# Autodesk Inventor assembly: Подъёмник
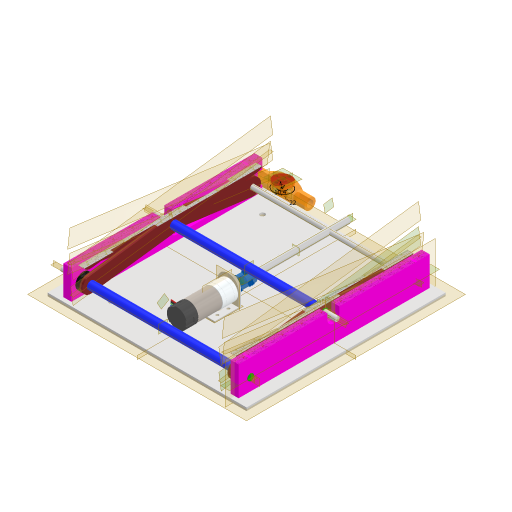
[picture p0: Inventor's stored thumbnail of the model, 512x512]
Saved by Autodesk Inventor 2023.2 (Build 272271030, 271C)
## iProperties
Created: 2025-03-18
Part Number: Подъёмник
Document SubType Name: Assembly
Designer: Коноваленко
Author: Коноваленко
## Documents named in this file (18)
- D:\!Rover\Rover\Rover_construction\Подъёмник.iam
- D:\!Rover\Rover\Rover_construction\Платформа подъёмника.ipt
- D:\!Rover\Rover\Rover_construction\Рельс платформы подъёмника.ipt
- D:\!Rover\Rover\Rover_construction\Рычаг платформы подъёмника.ipt
- D:\!Rover\Rover\Rover_construction\Основание подъёмника.ipt
- D:\!Rover\Rover\Rover_construction\Трубка.ipt
- D:\!Rover\Rover\Rover_construction\Рельс платформы подъёмника_MIR.ipt
- D:\!Rover\Rover\Rover_construction\Бабышка.ipt
- D:\!Rover\Rover\Rover_construction\Рельс платформы подъёмника_MIR1.ipt
- D:\!Rover\Rover\Rover_construction\Трубка основания.ipt
- D:\!Rover\Rover\Rover_construction\Подшипник.ipt
- D:\!Rover\Rover\Rover_construction\шпилька 6мм.ipt
- D:\!Rover\Rover\Rover_construction\Уголок крепления мотора.ipt
- D:\!Rover\Rover\Rover_construction\25d-metal-gearmotor-20.4-encoder.ipt
- D:\!Rover\Rover\Rover_construction\ftulka.ipt
- D:\!Rover\Rover\Rover_construction\Трапециевидный винт.ipt
- D:\!Rover\Rover\Rover_construction\Крепление ходовой гайки.ipt
- D:\!Rover\Rover\Rover_construction\THSL-300-8D õîäîâàÿ ãàéêà.ipt
## Components (53 placed, 17 different names)
1. Платформа подъёмника:1 — Совмещение:4, Заподлицо:4, Заподлицо:5, Заподлицо:10, Заподлицо:11, Совмещение:15
2. Рельс платформы подъёмника:1 — Совмещение:4, Заподлицо:4, Заподлицо:5, С поворотом:48, С поворотом:59
3. Основание подъёмника:1 — Совмещение:9, Заподлицо:8, Заподлицо:9, Заподлицо:12, Заподлицо:13, Совмещение:16, Совмещение:17, Заподлицо:14, Заподлицо:15, Совмещение:44, Заподлицо:21
4. Рельс платформы подъёмника:4 — Совмещение:9, Заподлицо:8, Заподлицо:9, С поворотом:32, Ползун:3, С поворотом:45, Совмещение:53
5. Трубка:1 — Жесткий:1, С поворотом:40, Совмещение:20, Совмещение:36, Заподлицо:16
6. Трубка:2 — С поворотом:38, С поворотом:39, Совмещение:18, Совмещение:39, Заподлицо:19
7. Рельс платформы подъёмника_MIR:1 — Заподлицо:10, Заподлицо:11, Совмещение:15, С поворотом:47, Ползун:5, Совмещение:53
8. Рельс платформы подъёмника_MIR1:1 — Заподлицо:12, Заподлицо:13, Совмещение:16, С поворотом:33, Ползун:4, С поворотом:46
9. Бабышка:9 — С поворотом:33, С поворотом:34
10. Бабышка:10 — С поворотом:32, С поворотом:37
11. Трубка основания:1 — Совмещение:30, Совмещение:31
12. Трубка основания:2 — Совмещение:18, Совмещение:19
13. Подшипник:1 — Ползун:5, С поворотом:55
14. Подшипник:2 — С поворотом:57
15. Подшипник:3 — Ползун:3, С поворотом:50
16. Подшипник:4 — Ползун:4, С поворотом:51
17. Трубка основания:3 — Совмещение:20, Совмещение:21
18. Трубка:3 — С поворотом:41, С поворотом:42, Совмещение:22, Совмещение:37, Заподлицо:17
19. Трубка:5 — С поворотом:43, С поворотом:44, Совмещение:24, Совмещение:38, Заподлицо:18
20. Трубка основания:4 — Совмещение:22, Совмещение:23
21. Трубка основания:5 — Совмещение:24, Совмещение:25
22. Трубка:6 — С поворотом:47, С поворотом:48, С поворотом:54
23. Трубка:7 — С поворотом:45, С поворотом:46, Совмещение:26, Совмещение:40, Заподлицо:20
24. Трубка основания:6 — Совмещение:28, Совмещение:29
25. Трубка основания:7 — Совмещение:26, Совмещение:27
26. шпилька 6мм:1 — С поворотом:50, С поворотом:51, С поворотом:52
27. Трубка:8 — С поворотом:52, С поворотом:53, Совмещение:28
28. Трубка:9 — С поворотом:56, С поворотом:58, Совмещение:30
29. шпилька 6мм:3 — С поворотом:55, С поворотом:56, С поворотом:57
30. Трубка:10 — С поворотом:59, Совмещение:32, Совмещение:35
31. Трубка основания:8 — Совмещение:32, Совмещение:33, Совмещение:34
32. Бабышка:11 — С поворотом:60
33. Бабышка:12 — С поворотом:61
34. шпилька 6мм:4 — Совмещение:37, Заподлицо:17
35. шпилька 6мм:5 — Совмещение:40, Заподлицо:20
36. шпилька 6мм:6 — Совмещение:38, Заподлицо:18
37. шпилька 6мм:7 — Совмещение:36, Заподлицо:16
38. шпилька 6мм:8 — Совмещение:34, Совмещение:35
39. шпилька 6мм:9 — Совмещение:39, Заподлицо:19
40. Уголок крепления мотора:1 — Совмещение:44, Заподлицо:21, Совмещение:45, Совмещение:46, Совмещение:47, Совмещение:52
41. 25d-metal-gearmotor-20.4-encoder:1 — Совмещение:45, Совмещение:46, Совмещение:47, Совмещение:49
42. ftulka:1 — Совмещение:49, Совмещение:50, Совмещение:51, Совмещение:52
43. Трапециевидный винт:6 — Совмещение:50, Совмещение:51
44. Крепление ходовой гайки:1 — Совмещение:54, Совмещение:55
45. THSL-300-8D õîäîâàÿ ãàéêà:1 — Совмещение:54, Совмещение:55
46. Рычаг платформы подъёмника:1 — С поворотом:11, С поворотом:36, С поворотом:37
47. Рычаг платформы подъёмника:2 — С поворотом:11, С поворотом:35, Жесткий:1, С поворотом:42, С поворотом:54
48. Рычаг платформы подъёмника:3 — С поворотом:8, С поворотом:17, Совмещение:21, Совмещение:25, Совмещение:31, С поворотом:61
49. Рычаг платформы подъёмника:4 — С поворотом:8, С поворотом:15, С поворотом:40, С поворотом:41, Совмещение:33
50. Рычаг платформы подъёмника:5 — С поворотом:12, С поворотом:35, С поворотом:58, С поворотом:60
51. Рычаг платформы подъёмника:6 — С поворотом:12, С поворотом:36, С поворотом:39, С поворотом:44, С поворотом:53
52. Рычаг платформы подъёмника:7 — С поворотом:16, С поворотом:17, С поворотом:38, С поворотом:43, Совмещение:29
53. Рычаг платформы подъёмника:8 — С поворотом:15, С поворотом:16, С поворотом:34, Совмещение:19, Совмещение:23, Совмещение:27
## Relationships (94: Mate 39, RevoluteJoint 35, Flush 16, TranslationJoint 3, WeldJoint 1)
- Совмещение:4 [Mate]: Платформа подъёмника:1 ↔ Рельс платформы подъёмника:1
- Совмещение:9 [Mate]: Основание подъёмника:1 ↔ Рельс платформы подъёмника:4
- Заподлицо:4 [Flush] (5 mm): Платформа подъёмника:1 ↔ Рельс платформы подъёмника:1
- Заподлицо:5 [Flush] (15 mm): Платформа подъёмника:1 ↔ Рельс платформы подъёмника:1
- Заподлицо:8 [Flush] (5 mm): Основание подъёмника:1 ↔ Рельс платформы подъёмника:4
- Заподлицо:9 [Flush] (15 mm): Основание подъёмника:1 ↔ Рельс платформы подъёмника:4
- Заподлицо:10 [Flush] (5 mm): Платформа подъёмника:1 ↔ Рельс платформы подъёмника_MIR:1
- Заподлицо:11 [Flush] (15 mm): Платформа подъёмника:1 ↔ Рельс платформы подъёмника_MIR:1
- Совмещение:15 [Mate]: Платформа подъёмника:1 ↔ Рельс платформы подъёмника_MIR:1
- С поворотом:8 [RevoluteJoint]: Рычаг платформы подъёмника:3 ↔ Рычаг платформы подъёмника:4
- С поворотом:11 [RevoluteJoint]: Рычаг платформы подъёмника:1 ↔ Рычаг платформы подъёмника:2
- С поворотом:12 [RevoluteJoint]: Рычаг платформы подъёмника:5 ↔ Рычаг платформы подъёмника:6
- С поворотом:15 [RevoluteJoint]: Рычаг платформы подъёмника:4 ↔ Рычаг платформы подъёмника:8
- С поворотом:16 [RevoluteJoint]: Рычаг платформы подъёмника:7 ↔ Рычаг платформы подъёмника:8
- С поворотом:17 [RevoluteJoint]: Рычаг платформы подъёмника:3 ↔ Рычаг платформы подъёмника:7
- Заподлицо:12 [Flush] (5 mm): Основание подъёмника:1 ↔ Рельс платформы подъёмника_MIR1:1
- Заподлицо:13 [Flush] (15 mm): Основание подъёмника:1 ↔ Рельс платформы подъёмника_MIR1:1
- Совмещение:16 [Mate]: Основание подъёмника:1 ↔ Рельс платформы подъёмника_MIR1:1
- Совмещение:17 [Mate]: Основание подъёмника:1
- Заподлицо:14 [Flush]: Основание подъёмника:1
- Заподлицо:15 [Flush]: Основание подъёмника:1
- С поворотом:32 [RevoluteJoint]: Рельс платформы подъёмника:4 ↔ Бабышка:10
- С поворотом:33 [RevoluteJoint]: Рельс платформы подъёмника_MIR1:1 ↔ Бабышка:9
- С поворотом:34 [RevoluteJoint]: Бабышка:9 ↔ Рычаг платформы подъёмника:8
- С поворотом:35 [RevoluteJoint]: Рычаг платформы подъёмника:2 ↔ Рычаг платформы подъёмника:5
- С поворотом:36 [RevoluteJoint]: Рычаг платформы подъёмника:1 ↔ Рычаг платформы подъёмника:6
- С поворотом:37 [RevoluteJoint]: Бабышка:10 ↔ Рычаг платформы подъёмника:1
- С поворотом:38 [RevoluteJoint] (-0.5 mm): Трубка:2 ↔ Рычаг платформы подъёмника:7
- С поворотом:39 [RevoluteJoint] (0.5 mm): Трубка:2 ↔ Рычаг платформы подъёмника:6
- Жесткий:1 [WeldJoint] (0.5 mm): Трубка:1 ↔ Рычаг платформы подъёмника:2
- С поворотом:40 [RevoluteJoint] (0.5 mm): Трубка:1 ↔ Рычаг платформы подъёмника:4
- Ползун:3 [TranslationJoint]: Рельс платформы подъёмника:4 ↔ Подшипник:3
- Ползун:4 [TranslationJoint]: Рельс платформы подъёмника_MIR1:1 ↔ Подшипник:4
- Совмещение:18 [Mate]: Трубка:2 ↔ Трубка основания:2
- Совмещение:19 [Mate] (0.5 mm): Трубка основания:2 ↔ Рычаг платформы подъёмника:8
- Совмещение:20 [Mate]: Трубка:1 ↔ Трубка основания:3
- Совмещение:21 [Mate] (0.5 mm): Трубка основания:3 ↔ Рычаг платформы подъёмника:3
- С поворотом:41 [RevoluteJoint] (0.5 mm): Трубка:3 ↔ Рычаг платформы подъёмника:4
- С поворотом:42 [RevoluteJoint] (-0.5 mm): Трубка:3 ↔ Рычаг платформы подъёмника:2
- С поворотом:43 [RevoluteJoint] (-0.5 mm): Трубка:5 ↔ Рычаг платформы подъёмника:7
- С поворотом:44 [RevoluteJoint] (-0.5 mm): Трубка:5 ↔ Рычаг платформы подъёмника:6
- Совмещение:22 [Mate]: Трубка:3 ↔ Трубка основания:4
- Совмещение:23 [Mate] (0.5 mm): Трубка основания:4 ↔ Рычаг платформы подъёмника:8
- Совмещение:24 [Mate]: Трубка:5 ↔ Трубка основания:5
- Совмещение:25 [Mate] (0.5 mm): Трубка основания:5 ↔ Рычаг платформы подъёмника:3
- С поворотом:45 [RevoluteJoint] (0.5 mm): Рельс платформы подъёмника:4 ↔ Трубка:7
- С поворотом:46 [RevoluteJoint] (0.5 mm): Рельс платформы подъёмника_MIR1:1 ↔ Трубка:7
- Совмещение:26 [Mate]: Трубка:7 ↔ Трубка основания:7
- Совмещение:27 [Mate] (0.5 mm): Трубка основания:7 ↔ Рычаг платформы подъёмника:8
- С поворотом:47 [RevoluteJoint] (0.5 mm): Рельс платформы подъёмника_MIR:1 ↔ Трубка:6
- С поворотом:48 [RevoluteJoint] (-0.5 mm): Рельс платформы подъёмника:1 ↔ Трубка:6
- Ползун:5 [TranslationJoint]: Рельс платформы подъёмника_MIR:1 ↔ Подшипник:1
- С поворотом:50 [RevoluteJoint]: Подшипник:3 ↔ шпилька 6мм:1
- С поворотом:51 [RevoluteJoint]: Подшипник:4 ↔ шпилька 6мм:1
- С поворотом:52 [RevoluteJoint]: шпилька 6мм:1 ↔ Трубка:8
- С поворотом:53 [RevoluteJoint] (-0.5 mm): Трубка:8 ↔ Рычаг платформы подъёмника:6
- С поворотом:54 [RevoluteJoint] (-11.5 mm): Трубка:6 ↔ Рычаг платформы подъёмника:2
- Совмещение:28 [Mate]: Трубка основания:6 ↔ Трубка:8
- Совмещение:29 [Mate] (0.5 mm): Трубка основания:6 ↔ Рычаг платформы подъёмника:7
- С поворотом:55 [RevoluteJoint]: Подшипник:1 ↔ шпилька 6мм:3
- С поворотом:56 [RevoluteJoint]: Трубка:9 ↔ шпилька 6мм:3
- С поворотом:57 [RevoluteJoint]: Подшипник:2 ↔ шпилька 6мм:3
- С поворотом:58 [RevoluteJoint] (-4.5 mm): Трубка:9 ↔ Рычаг платформы подъёмника:5
- Совмещение:30 [Mate]: Трубка основания:1 ↔ Трубка:9
- Совмещение:31 [Mate] (0.5 mm): Трубка основания:1 ↔ Рычаг платформы подъёмника:3
- С поворотом:59 [RevoluteJoint] (-0.5 mm): Рельс платформы подъёмника:1 ↔ Трубка:10
- Совмещение:32 [Mate]: Трубка:10 ↔ Трубка основания:8
- Совмещение:33 [Mate] (0.5 mm): Трубка основания:8 ↔ Рычаг платформы подъёмника:4
- С поворотом:60 [RevoluteJoint] (-4.5 mm): Бабышка:11 ↔ Рычаг платформы подъёмника:5
- С поворотом:61 [RevoluteJoint] (-0.5 mm): Бабышка:12 ↔ Рычаг платформы подъёмника:3
- Совмещение:34 [Mate]: Трубка основания:8 ↔ шпилька 6мм:8
- Совмещение:35 [Mate] (-4.5 mm): Трубка:10 ↔ шпилька 6мм:8
- Совмещение:36 [Mate]: Трубка:1 ↔ шпилька 6мм:7
- Заподлицо:16 [Flush] (-15.5 mm): Трубка:1 ↔ шпилька 6мм:7
- Совмещение:37 [Mate]: Трубка:3 ↔ шпилька 6мм:4
- Заподлицо:17 [Flush] (-15.5 mm): Трубка:3 ↔ шпилька 6мм:4
- Совмещение:38 [Mate]: Трубка:5 ↔ шпилька 6мм:6
- Заподлицо:18 [Flush] (-15.5 mm): Трубка:5 ↔ шпилька 6мм:6
- Совмещение:39 [Mate]: Трубка:2 ↔ шпилька 6мм:9
- Заподлицо:19 [Flush] (-15.5 mm): Трубка:2 ↔ шпилька 6мм:9
- Совмещение:40 [Mate]: Трубка:7 ↔ шпилька 6мм:5
- Заподлицо:20 [Flush] (-15.5 mm): Трубка:7 ↔ шпилька 6мм:5
- Совмещение:44 [Mate]: Основание подъёмника:1 ↔ Уголок крепления мотора:1
- Заподлицо:21 [Flush]: Основание подъёмника:1 ↔ Уголок крепления мотора:1
- Совмещение:45 [Mate]: Уголок крепления мотора:1 ↔ 25d-metal-gearmotor-20.4-encoder:1
- Совмещение:46 [Mate]: Уголок крепления мотора:1 ↔ 25d-metal-gearmotor-20.4-encoder:1
- Совмещение:47 [Mate]: Уголок крепления мотора:1 ↔ 25d-metal-gearmotor-20.4-encoder:1
- Совмещение:49 [Mate]: 25d-metal-gearmotor-20.4-encoder:1 ↔ ftulka:1
- Совмещение:50 [Mate]: ftulka:1 ↔ Трапециевидный винт:6
- Совмещение:51 [Mate] (-10 mm): ftulka:1 ↔ Трапециевидный винт:6
- Совмещение:52 [Mate] (2 mm): Уголок крепления мотора:1 ↔ ftulka:1
- Совмещение:53 [Mate]: Рельс платформы подъёмника:4 ↔ Рельс платформы подъёмника_MIR:1
- Совмещение:54 [Mate]: Крепление ходовой гайки:1 ↔ THSL-300-8D õîäîâàÿ ãàéêà:1
- Совмещение:55 [Mate]: Крепление ходовой гайки:1 ↔ THSL-300-8D õîäîâàÿ ãàéêà:1
